# Autodesk Inventor assembly: 付け根_1
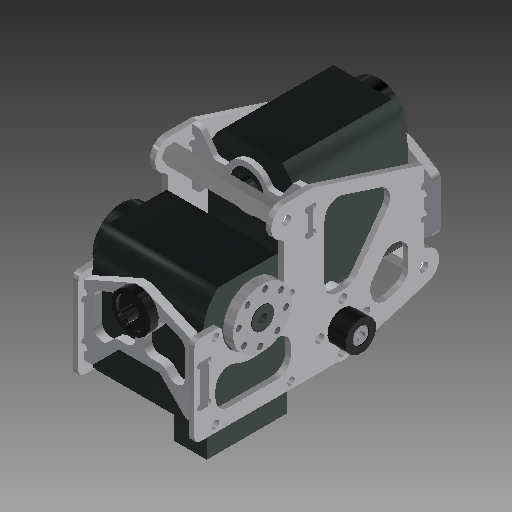
[picture p0: Inventor's stored thumbnail of the model, 512x512]
Saved by Autodesk Inventor 2018 (Build 220112000, 112)
## iProperties
Created: 2016-04-27
Part Number: 付け根_1
Document SubType Name: Assembly
Designer: hiroaki
Mass: 277.749 g
Surface Area: 481.209 cm^2
Volume: 134.062 cm^3
Density: 2.07179 g/cm^3
Author: hiroaki
## Documents named in this file (15)
- C:\Users\taka\Documents\github\OpenPlatform\mechanism\OpenPlatform_ver3_0\下半身_160823\付け根\付け根_1_MIR.iam
- C:\Users\taka\Documents\github\OpenPlatform\mechanism\OpenPlatform_ver3_0\既製品\B3M11xx.ipt
- C:\Users\taka\Documents\github\OpenPlatform\mechanism\OpenPlatform_ver3_0\既製品\free_horn.ipt
- C:\Users\taka\Documents\github\OpenPlatform\mechanism\OpenPlatform_ver3_0\下半身_160823\付け根\付け根_サブフレーム_1_2.ipt
- C:\Users\taka\Documents\github\OpenPlatform\mechanism\OpenPlatform_ver3_0\下半身\リンク\スペーサ\付け根_フリー軸_1_1.ipt
- C:\Users\taka\Documents\github\OpenPlatform\mechanism\OpenPlatform_ver3_0\既製品\ASU-340.ipt
- C:\Users\taka\Documents\github\OpenPlatform\mechanism\OpenPlatform_ver3_0\下半身_160823\付け根\付け根_メインフレーム_6_1.ipt
- C:\Users\taka\Documents\github\OpenPlatform\mechanism\OpenPlatform_ver3_0\下半身_160823\付け根\付け根_サブフレーム_1_4.ipt
- C:\Users\taka\Documents\github\OpenPlatform\mechanism\OpenPlatform_ver3_0\下半身_160823\付け根\付け根_サブフレーム_6_2.ipt
- C:\Users\taka\Documents\github\OpenPlatform\mechanism\OpenPlatform_ver3_0\既製品\新規購入\BRU-305_5.ipt
- C:\Users\taka\Documents\github\OpenPlatform\mechanism\OpenPlatform_ver3_0\下半身_160823\付け根\付け根_メインフレーム_2_1.ipt
- C:\Users\taka\Documents\github\OpenPlatform\mechanism\OpenPlatform_ver3_0\下半身_160823\付け根\付け根_メインフレーム_2_1_MIR.ipt
- C:\Users\taka\Documents\github\OpenPlatform\mechanism\OpenPlatform_ver3_0\下半身_160823\付け根\付け根_サブフレーム_1_3.ipt
- C:\Users\taka\Documents\github\OpenPlatform\mechanism\OpenPlatform_ver3_0\既製品\新規購入\BRU-306_5.ipt
- C:\Users\taka\Documents\github\OpenPlatform\mechanism\OpenPlatform_ver3_0\下半身_160823\付け根\付け根_サブフレーム_6_4.ipt
## Components (19 placed, 14 different names)
1. free_horn:1 — 挿入:1
2. B3M11xx:3 — 挿入:1, 挿入:50, 挿入:51, 挿入:53, 挿入:54, メイト:2
3. B3M11xx:4 — 挿入:7, 挿入:8, 角度:2, 挿入:41, 挿入:42, 角度:4
4. 付け根_サブフレーム_1_2:1 — 挿入:7, 挿入:8, メイト:5
5. 付け根_フリー軸_1_1:1 — 挿入:58, 挿入:59
6. 付け根_フリー軸_1_1:2 — 挿入:56, 挿入:57
7. ASU-340:1 — 挿入:52, 角度:4
8. ASU-340:2 — 角度:2, 挿入:60
9. 付け根_メインフレーム_6_1:1 — 挿入:41, 挿入:42, 挿入:45, 角度:3, メイト:1, メイト:6
10. 付け根_サブフレーム_1_4:1 — 挿入:55
11. 付け根_サブフレーム_6_2:1 — 挿入:46
12. BRU-305_5:1 — 挿入:45, 挿入:46
13. 付け根_メインフレーム_2_1:1 — 挿入:53, 挿入:54, 角度:3, メイト:1, メイト:4, 挿入:58, 挿入:59, メイト:5, 挿入:66, メイト:6
14. 付け根_メインフレーム_2_1_MIR:1 — 挿入:50, 挿入:51, 挿入:52, メイト:3, 挿入:56, 挿入:57, 挿入:60, 挿入:63
15. 付け根_サブフレーム_1_3:1 — メイト:2, メイト:3, メイト:4, 挿入:55
16. BRU-306_5:1 — 挿入:63
17. 付け根_サブフレーム_6_4:1
18. BRU-306_5:2 — 挿入:66
19. 付け根_サブフレーム_6_4:2
## Relationships (31: Insert 22, Mate 6, Angle 3)
- 挿入:1 [Insert]: free_horn:1 ↔ B3M11xx:3
- 挿入:7 [Insert]: B3M11xx:4 ↔ 付け根_サブフレーム_1_2:1
- 挿入:8 [Insert]: B3M11xx:4 ↔ 付け根_サブフレーム_1_2:1
- 角度:2 [Angle] (0 deg): B3M11xx:4 ↔ ASU-340:2
- 挿入:41 [Insert]: B3M11xx:4 ↔ 付け根_メインフレーム_6_1:1
- 挿入:42 [Insert]: B3M11xx:4 ↔ 付け根_メインフレーム_6_1:1
- 挿入:45 [Insert]: 付け根_メインフレーム_6_1:1 ↔ BRU-305_5:1
- 挿入:46 [Insert]: 付け根_サブフレーム_6_2:1 ↔ BRU-305_5:1
- 挿入:50 [Insert]: B3M11xx:3 ↔ 付け根_メインフレーム_2_1_MIR:1
- 挿入:51 [Insert]: B3M11xx:3 ↔ 付け根_メインフレーム_2_1_MIR:1
- 挿入:52 [Insert]: ASU-340:1 ↔ 付け根_メインフレーム_2_1_MIR:1
- 挿入:53 [Insert]: B3M11xx:3 ↔ 付け根_メインフレーム_2_1:1
- 挿入:54 [Insert]: B3M11xx:3 ↔ 付け根_メインフレーム_2_1:1
- 角度:3 [Angle] (0 deg): 付け根_メインフレーム_6_1:1 ↔ 付け根_メインフレーム_2_1:1
- メイト:1 [Mate]: 付け根_メインフレーム_6_1:1 ↔ 付け根_メインフレーム_2_1:1
- メイト:2 [Mate]: B3M11xx:3 ↔ 付け根_サブフレーム_1_3:1
- メイト:3 [Mate]: 付け根_メインフレーム_2_1_MIR:1 ↔ 付け根_サブフレーム_1_3:1
- メイト:4 [Mate] (0.025 mm): 付け根_メインフレーム_2_1:1 ↔ 付け根_サブフレーム_1_3:1
- 挿入:55 [Insert]: 付け根_サブフレーム_1_4:1 ↔ 付け根_サブフレーム_1_3:1
- 挿入:56 [Insert]: 付け根_フリー軸_1_1:2 ↔ 付け根_メインフレーム_2_1_MIR:1
- 挿入:57 [Insert]: 付け根_フリー軸_1_1:2 ↔ 付け根_メインフレーム_2_1_MIR:1
- 挿入:58 [Insert]: 付け根_フリー軸_1_1:1 ↔ 付け根_メインフレーム_2_1:1
- 挿入:59 [Insert]: 付け根_フリー軸_1_1:1 ↔ 付け根_メインフレーム_2_1:1
- メイト:5 [Mate]: 付け根_サブフレーム_1_2:1 ↔ 付け根_メインフレーム_2_1:1
- 挿入:60 [Insert]: ASU-340:2 ↔ 付け根_メインフレーム_2_1_MIR:1
- [Insert]: BRU-306_5:1 ↔ 付け根_サブフレーム_6_4:1
- 挿入:63 [Insert]: 付け根_メインフレーム_2_1_MIR:1 ↔ BRU-306_5:1
- [Insert]: BRU-306_5:2 ↔ 付け根_サブフレーム_6_4:2
- 挿入:66 [Insert]: 付け根_メインフレーム_2_1:1 ↔ BRU-306_5:2
- 角度:4 [Angle] (90 deg): B3M11xx:4 ↔ ASU-340:1
- メイト:6 [Mate] (0.005 mm): 付け根_メインフレーム_6_1:1 ↔ 付け根_メインフレーム_2_1:1
## Named parameters: d139_d143 = 0 mm
